# Autodesk Inventor assembly: Neo550OnVersa2Stage
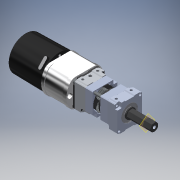
[picture p0: Inventor's stored thumbnail of the model, 180x180]
Saved by Autodesk Inventor 2018.3 (Build 223284000, 284)
## iProperties
Created: 2016-10-31
Part Number: Neo550OnVersa2Stage
Description: STEP AP214
Document SubType Name: Assembly
Designer: user
Mass: 698.532 g
Surface Area: 781.615 cm^2
Volume: 185.532 cm^3
Density: 3.76503 g/cm^3
Sending System: SolidWorks 2016
Preprocessor: SwSTEP 2.0
Title: 217-4973_2stage_BAG.STEP
Revision Number: ANY
## Documents named in this file (18)
- C:\Users\myerpaul\Documents\GrabCAD\Infinite Recharge 2020\Build season\180 VERSAPLANETARY\Neo550OnVersa2Stage.iam
- C:\Users\myerpaul\Documents\GrabCAD\Infinite Recharge 2020\Build season\180 VERSAPLANETARY\217-2625-026 Rev1.ipt
- C:\Users\myerpaul\Documents\GrabCAD\Infinite Recharge 2020\Build season\180 VERSAPLANETARY\217-2742-001 Rev4.ipt
- C:\Users\myerpaul\Documents\GrabCAD\Infinite Recharge 2020\Build season\180 VERSAPLANETARY\217-2625-017 Rev1_9714K61.ipt
- C:\Users\myerpaul\Documents\GrabCAD\Infinite Recharge 2020\Build season\180 VERSAPLANETARY\217-2625-003 Rev1.ipt
- C:\Users\myerpaul\Documents\GrabCAD\Infinite Recharge 2020\Build season\180 VERSAPLANETARY\217-2625-018 Rev1_98541A410.ipt
- C:\Users\myerpaul\Documents\GrabCAD\Infinite Recharge 2020\Build season\180 VERSAPLANETARY\832-2250-Base-Kit-Screw_SSA0832-0500ZC.ipt
- C:\Users\myerpaul\Documents\GrabCAD\Infinite Recharge 2020\Build season\180 VERSAPLANETARY\217-2625-025 Rev1.ipt
- C:\Users\myerpaul\Documents\GrabCAD\Infinite Recharge 2020\Build season\180 VERSAPLANETARY\217-4649-002 Rev1_SSA0832-0500ZC.ipt
- C:\Users\myerpaul\Documents\GrabCAD\Infinite Recharge 2020\Build season\180 VERSAPLANETARY\217-4649-006 Rev1_SSA0004-008BA.ipt
- C:\Users\myerpaul\Documents\GrabCAD\Infinite Recharge 2020\Build season\180 VERSAPLANETARY\217-2820 Rev1_Public.iam
- C:\Users\myerpaul\Documents\GrabCAD\Infinite Recharge 2020\Build season\180 VERSAPLANETARY\217-2816-001 Rev1.ipt
- C:\Users\myerpaul\Documents\GrabCAD\Infinite Recharge 2020\Build season\180 VERSAPLANETARY\217-4649-001 Rev1.ipt
- C:\Users\myerpaul\Documents\GrabCAD\Infinite Recharge 2020\Build season\180 VERSAPLANETARY\217-4649-007 Rev1_94105A824.ipt
- C:\Users\myerpaul\Documents\GrabCAD\Infinite Recharge 2020\Build season\180 VERSAPLANETARY\217-2625-011 Rev1.ipt
- C:\Users\myerpaul\Documents\GrabCAD\Infinite Recharge 2020\Build season\180 VERSAPLANETARY\217-2822-002 Rev4.ipt
- C:\Users\myerpaul\Documents\GrabCAD\Infinite Recharge 2020\Build season\180 VERSAPLANETARY\NEO_Adapter_Fixed.ipt
- C:\Users\myerpaul\Documents\GrabCAD\Infinite Recharge 2020\Build season\180 VERSAPLANETARY\REV-21-1650.ipt
## Components (23 placed, 22 different names)
1. 217-2625-026 Rev1_1
2. 217-2742-001 Rev4_2
3. 217-2742-001 Rev4_3
4. 217-2625-017 Rev1_9714K61_4
5. 217-2625-003 Rev1_5
6. 217-2625-018 Rev1_98541A410_6
7. 832-2250-Base-Kit-Screw_SSA0832-0500ZC_7
8. 832-2250-Base-Kit-Screw_SSA0832-0500ZC_8 — Mate:1
9. 217-2625-025 Rev1_9 — Angle:1
10. 217-4649-002 Rev1_SSA0832-0500ZC_10
11. 217-4649-002 Rev1_SSA0832-0500ZC_11
12. 217-2820 Rev1_Public_16 [sub-assembly]
13. 217-2816-001 Rev1_17
14. 217-2820 Rev1_Public_18 [sub-assembly]
15. 217-2816-001 Rev1_19
16. 217-4649-001 Rev1_20
17. 217-4649-007 Rev1_94105A824_21
18. 217-2625-011 Rev1_22
19. 217-4649-006 Rev1_SSA0004-008BA:1
20. 217-4649-006 Rev1_SSA0004-008BA:2
21. 217-2822-002 Rev4:1 — Mate:2
22. NEO_Adapter_Fixed:1 — Mate:1, Angle:1, Mate:2, Insert:1
23. REV-21-1650:1 — Insert:1
## Relationships (4: Mate 2, Angle 1, Insert 1)
- Mate:1: 832-2250-Base-Kit-Screw_SSA0832-0500ZC_8 ↔ NEO_Adapter_Fixed:1
- Angle:1 (0 deg): 217-2625-025 Rev1_9 ↔ NEO_Adapter_Fixed:1
- Mate:2: 217-2822-002 Rev4:1 ↔ NEO_Adapter_Fixed:1
- Insert:1: NEO_Adapter_Fixed:1 ↔ REV-21-1650:1
